# Autodesk Inventor assembly: Rb oven housing
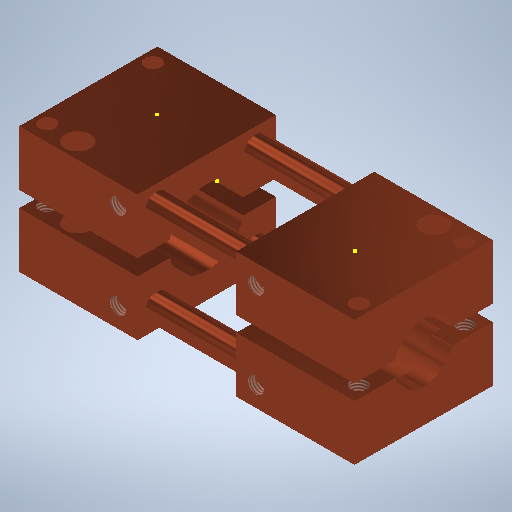
[picture p0: Inventor's stored thumbnail of the model, 512x512]
Saved by Autodesk Inventor 2025.1 (Build 291241000, 241)
## iProperties
Created: 2025-04-24
Part Number: Rb oven housing
Document SubType Name: Assembly
Designer: E. Moreno
Author: E. Moreno
Title: Carcasa Horno - Ensamblado
## Documents named in this file (3)
- C:\Users\dell 5810\Documents\M\GitHub\LAFriOC\Rb oven\Rb oven housing\Modificación\Rb oven housing.iam
- C:\Users\dell 5810\Documents\M\GitHub\LAFriOC\Rb oven\Rb oven housing\Modificación\Rb oven housing - Bottom.iam
- C:\Users\dell 5810\Documents\M\GitHub\LAFriOC\Rb oven\Rb oven housing\Modificación\Rb oven housing - Top.iam
## Components (2 placed, 2 different names)
1. Rb oven housing - Bottom:1 [sub-assembly] — Coincidencia:1, Coincidencia:2
2. Rb oven housing - Top:1 [sub-assembly] — Coincidencia:1, Coincidencia:2
## Relationships (2: Mate 2)
- Coincidencia:1 [Mate] (18 mm): Rb oven housing - Bottom:1 ↔ Rb oven housing - Top:1
- Coincidencia:2 [Mate]: Rb oven housing - Bottom:1 ↔ Rb oven housing - Top:1
